# Autodesk Inventor assembly: CNC3
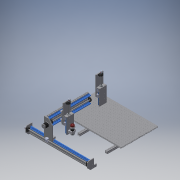
[picture p0: Inventor's stored thumbnail of the model, 180x180]
Saved by Autodesk Inventor 2018 (Build 220112000, 112)
## iProperties
Created: 2018-10-09
Part Number: CNC3
Material: Genérico
Document SubType Name: Assembly
Designer: Georgines
Author: Georgines
## Documents named in this file (29)
- C:\Users\Usuário\Documents\OpenCNC\MONTAGEM\CNC3.iam
- C:\Users\Usuário\Documents\OpenCNC\COMPONENTES_MECANICOS\BLOCOS_GUIAS_LINEARES\SBR16UU.ipt
- C:\Users\Usuário\Documents\OpenCNC\MONTAGEM\CNC1\APOIO_PERFIL_STRUTURAL.ipt
- C:\Users\Usuário\Documents\OpenCNC\MONTAGEM\CNC1\LATERAL_BLOCOS_BASE.ipt
- C:\Users\Usuário\Documents\OpenCNC\MONTAGEM\BLOCO_SUPORTE_EIXO_Z.ipt
- C:\Users\Usuário\Documents\OpenCNC\BAIXADOS\spindle-bldc-500w-1.snapshot.1\SPINDLE_500WSpindle.iam
- C:\Users\Usuário\Documents\OpenCNC\BAIXADOS\spindle-bracket-1.snapshot.2\SUPORTE_SPINDLESpindle Bracket.ipt
- C:\Users\Usuário\Documents\OpenCNC\MONTAGEM\CNC1\BLOCO_SUPORTE_SPINDLE.ipt
- C:\Users\Usuário\Documents\OpenCNC\BAIXADOS\bearing-support-unit-1.snapshot.1\BK12BK12.ipt
- C:\Users\Usuário\Documents\OpenCNC\BAIXADOS\bearing-support-unit-1.snapshot.1\BF12.ipt
- C:\Users\Usuário\Documents\OpenCNC\COMPONENTES_MECANICOS\GUIAS_LINEARES\SBR16_200MM.ipt
- C:\Users\Usuário\Documents\OpenCNC\COMPONENTES_MECANICOS\GUIAS_LINEARES\SBR16_EIXO_X_1.ipt
- C:\Users\Usuário\Documents\OpenCNC\BAIXADOS\stepper motor NEMA 23 57x76.ipt
- C:\Users\Usuário\Documents\OpenCNC\MONTAGEM\CHAPA_APOIO_CASTANHA_EIXO_Z.ipt
- C:\Users\Usuário\Documents\OpenCNC\COMPONENTES_MECANICOS\GUIAS_LINEARES\SBR16_EIXO_Y_1.ipt
- C:\Users\Usuário\Documents\OpenCNC\COMPONENTES_MECANICOS\PERFIL_ESTRUTURAL\PERFIL_ESTRUTURAL_40X80_EIXO_Y.ipt
- C:\Users\Usuário\Documents\OpenCNC\COMPONENTES_MECANICOS\PERFIL_ESTRUTURAL\PERFIL_ESTRUTURAL_40X40_EIXO_Y_PERPENDICULAR.ipt
- C:\Users\Usuário\Documents\OpenCNC\COMPONENTES_MECANICOS\FUSOS\SFU16XX_Y1.ipt
- C:\Users\Usuário\Documents\OpenCNC\COMPONENTES_MECANICOS\FUSOS\SFU16XX_Z.ipt
- C:\Users\Usuário\Documents\OpenCNC\COMPONENTES_MECANICOS\FUSOS\SFU16XX_X.ipt
- C:\Users\Usuário\Documents\OpenCNC\COMPONENTES_MECANICOS\CASTANHAS\CASTANHA_SFU1604SFU1604.ipt
- C:\Users\Usuário\Documents\OpenCNC\COMPONENTES_MECANICOS\ACOPLADORES\ACLOPLADOR_Jaw 6,35x10 d=25 L=30.ipt
- C:\Users\Usuário\Documents\OpenCNC\COMPONENTES_MECANICOS\PERFIL_ESTRUTURAL\PERFIL_ESTRUTURAL_30X60_EIXO_X1.ipt
- C:\Users\Usuário\Documents\OpenCNC\COMPONENTES_MECANICOS\PERFIL_ESTRUTURAL\PERFIL_ESTRUTURAL_30X60_EIXO_X2.ipt
- C:\Users\Usuário\Documents\OpenCNC\COMPONENTES_MECANICOS\SUPORTE_CASTANHAS\SUPORTE_CASTANHAS_DSG16H.ipt
- C:\Users\Usuário\Documents\OpenCNC\MONTAGEM\SUPORTE_MANCAL_FRONTAL.ipt
- C:\Users\Usuário\Documents\OpenCNC\COMPONENTES_MECANICOS\PERFIL_ESTRUTURAL\PERFIL_ESTRUTURAL_20X40_MESA.ipt
- C:\Users\Usuário\Documents\BLOCO_SUPORTE_SPINDLE_E_EIXO_X.ipt
- C:\Users\Usuário\Documents\OpenCNC\MONTAGEM\SUPORTE_MANCAL_TRASEIRO.ipt
## Components (81 placed, 28 different names)
1. SBR16UU:1 — ALINHAMENTO_BOCOS_BASE_4, Alinhamento:32, Coincidência:22, Coincidência:109, Alinhamento:277, Alinhamento:278
2. SBR16UU:2 — ALINHAMENTO_BOCOS_BASE_4, Alinhamento:31, Alinhamento:149, Coincidência:110
3. APOIO_PERFIL_STRUTURAL:1 — Alinhamento:31, Alinhamento:32, Coincidência:22, Alinhamento:85, Alinhamento:149, Alinhamento:177, Coincidência:253, Alinhamento:277, Alinhamento:278
4. LATERAL_BLOCOS_BASE:1 — Alinhamento:85, Alinhamento:177, Coincidência:173, Alinhamento:191, Alinhamento:192, Coincidência:191, Ângulo:3, Alinhamento:200, Ângulo:9, Coincidência:198, Alinhamento:208, Coincidência:253, Alinhamento:275, Alinhamento:276
5. BLOCO_SUPORTE_EIXO_Z:1 — Coincidência:66, Coincidência:77, Alinhamento:118, Alinhamento:122, Alinhamento:124, Coincidência:232, Alinhamento:253, Alinhamento:254
6. SPINDLE_500WSpindle:1 [sub-assembly] — Coincidência:63, Alinhamento:99
7. SUPORTE_SPINDLESpindle Bracket:1 — Coincidência:62, Alinhamento:97, Alinhamento:98, Coincidência:63, Alinhamento:99
8. BLOCO_SUPORTE_SPINDLE:1 — Coincidência:62, Alinhamento:97, Alinhamento:98, Coincidência:79, Coincidência:81, Alinhamento:119, Alinhamento:120, Alinhamento:121, Alinhamento:151, Alinhamento:152, Alinhamento:153
9. BK12BK12:1 — Coincidência:66, Alinhamento:103, Alinhamento:124, Coincidência:181, Coincidência:182, Coincidência:203
10. BF12:1 — Alinhamento:103, Coincidência:180, Coincidência:184, Coincidência:234
11. SBR16UU:9 — Alinhamento:104, Alinhamento:106, Alinhamento:109, Coincidência:75, Coincidência:76, Coincidência:77, Coincidência:78, Alinhamento:122
12. SBR16UU:10 — Alinhamento:104, Alinhamento:107, Alinhamento:108, Alinhamento:109, Coincidência:76, Coincidência:80, Coincidência:234
13. SBR16UU:11 — Alinhamento:105, Alinhamento:106, Alinhamento:110, Coincidência:75
14. SBR16UU:12 — Alinhamento:105, Alinhamento:107, Alinhamento:108, Alinhamento:110, Alinhamento:118
15. SBR16_200MM:1 — Coincidência:78, Coincidência:79, Alinhamento:119, Alinhamento:121
16. SBR16_200MM:2 — Coincidência:80, Coincidência:81, Alinhamento:120
17. SBR16UU:13 — Coincidência:169, Alinhamento:194, Alinhamento:252
18. SBR16UU:14 — Coincidência:168, Alinhamento:190, Alinhamento:195, Alinhamento:249, Alinhamento:250, Alinhamento:251
19. SBR16UU:15 — Alinhamento:173, Coincidência:166, Alinhamento:190, Alinhamento:195
20. stepper motor NEMA 23 57x76:1 — Coincidência:187, Coincidência:188, Coincidência:198, Ângulo:12
21. CHAPA_APOIO_CASTANHA_EIXO_Z:1 — Alinhamento:151, Alinhamento:152, Alinhamento:153, Coincidência:177, Ângulo:1
22. SBR16_EIXO_Y_1:1 — Coincidência:109, Coincidência:110, Coincidência:115, Alinhamento:158, Alinhamento:159, Alinhamento:280
23. PERFIL_ESTRUTURAL_40X80_EIXO_Y:1 — Coincidência:115, Alinhamento:158, Alinhamento:159, Alinhamento:165, Alinhamento:166, Ângulo:9, Alinhamento:203, Alinhamento:205, Alinhamento:279, Coincidência:254, Coincidência:255, Coincidência:256, Alinhamento:283
24. PERFIL_ESTRUTURAL_40X40_EIXO_Y_PERPENDICULAR:1 — Coincidência:210, Alinhamento:247
25. PERFIL_ESTRUTURAL_40X40_EIXO_Y_PERPENDICULAR:2 — Alinhamento:165, Alinhamento:167, Alinhamento:283
26. PERFIL_ESTRUTURAL_40X40_EIXO_Y_PERPENDICULAR:3 — Alinhamento:166, Alinhamento:167
27. stepper motor NEMA 23 57x76:3 — Coincidência:159, Coincidência:160
28. SBR16UU:17 — Alinhamento:173, Coincidência:167, Alinhamento:194, Alinhamento:257
29. SFU16XX_Y1:1 — Coincidência:136, Coincidência:137, Coincidência:138, Coincidência:139, Coincidência:152, Coincidência:155, Coincidência:157
30. SFU16XX_Z:1 — Coincidência:178, Coincidência:179, Coincidência:180, Coincidência:181, Coincidência:182, Coincidência:183, Coincidência:184
31. SFU16XX_X:1 — Coincidência:146, Coincidência:148, Coincidência:149, Coincidência:151, Coincidência:154, Coincidência:175, Coincidência:176
32. BK12BK12:2 — Coincidência:136, Coincidência:137, Alinhamento:178, Ângulo:21
33. BF12:2 — Coincidência:138, Coincidência:139, Alinhamento:178, Alinhamento:203, Coincidência:205, Ângulo:20
34. BK12BK12:4 — Coincidência:146, Alinhamento:180, Coincidência:151, Ângulo:12, Alinhamento:275, Alinhamento:276
35. BF12:4 — Coincidência:148, Coincidência:149, Alinhamento:180, Ângulo:14, Alinhamento:212
36. CASTANHA_SFU1604SFU1604:1 — Coincidência:152, Coincidência:189, Coincidência:190, Ângulo:2
37. CASTANHA_SFU1604SFU1604:3 — Coincidência:154, Coincidência:195, Coincidência:196
38. CASTANHA_SFU1604SFU1604:4 — Coincidência:177, Coincidência:178, Ângulo:1, Coincidência:203
39. ACLOPLADOR_Jaw 6,35x10 d=25 L=30:2 — Coincidência:155, Coincidência:157, Coincidência:159, Coincidência:160
40. ACLOPLADOR_Jaw 6,35x10 d=25 L=30:3 — Coincidência:179, Coincidência:183
41. ACLOPLADOR_Jaw 6,35x10 d=25 L=30:4 — Coincidência:175, Coincidência:176, Coincidência:187, Coincidência:188
42. PERFIL_ESTRUTURAL_30X60_EIXO_X1:1 — Coincidência:163, Alinhamento:183, Alinhamento:184, Alinhamento:187, Alinhamento:188, Coincidência:173, Alinhamento:191, Alinhamento:192, Coincidência:207, Alinhamento:209, Alinhamento:210
43. PERFIL_ESTRUTURAL_30X60_EIXO_X2:1 — Coincidência:164, Alinhamento:185, Alinhamento:186, Alinhamento:187, Alinhamento:188, Coincidência:208, Alinhamento:211
44. SBR16_EIXO_X_1:2 — Coincidência:163, Alinhamento:183, Alinhamento:184, Coincidência:168, Coincidência:169, Ângulo:14
45. SBR16_EIXO_X_1:3 — Coincidência:164, Alinhamento:185, Alinhamento:186, Coincidência:166, Coincidência:167
46. SUPORTE_CASTANHAS_DSG16H:1 — Coincidência:189, Coincidência:190, Ângulo:2, Coincidência:191, Ângulo:3, Alinhamento:200, Coincidência:205, Alinhamento:208
47. SUPORTE_CASTANHAS_DSG16H:3 — Coincidência:195, Coincidência:196, Coincidência:233, Alinhamento:256
48. SUPORTE_MANCAL_FRONTAL:1 — Alinhamento:205, Coincidência:211, Alinhamento:247, Alinhamento:279, Alinhamento:280, Ângulo:20, Alinhamento:281, Alinhamento:282
49. PERFIL_ESTRUTURAL_30X60_EIXO_X1:2 — Coincidência:207, Alinhamento:209, Alinhamento:210, Coincidência:208, Alinhamento:211, Alinhamento:212
50. PERFIL_ESTRUTURAL_20X40_MESA:1 — Coincidência:209, Coincidência:210, Coincidência:211, Alinhamento:213, Alinhamento:214
51. PERFIL_ESTRUTURAL_20X40_MESA:2 — Coincidência:209, Alinhamento:213, Alinhamento:214, Alinhamento:215, Alinhamento:216, Coincidência:213
52. PERFIL_ESTRUTURAL_20X40_MESA:3 — Alinhamento:215, Alinhamento:216, Coincidência:213, Coincidência:214, Alinhamento:217, Alinhamento:218
53. PERFIL_ESTRUTURAL_20X40_MESA:4 — Coincidência:214, Coincidência:215, Alinhamento:217, Alinhamento:218, Coincidência:216, Alinhamento:219, Alinhamento:220
54. PERFIL_ESTRUTURAL_20X40_MESA:5 — Coincidência:215, Coincidência:216, Alinhamento:219, Alinhamento:220, Coincidência:217, Alinhamento:221, Alinhamento:222
55. PERFIL_ESTRUTURAL_20X40_MESA:6 — Coincidência:217, Alinhamento:221, Alinhamento:222, Coincidência:218, Alinhamento:223, Alinhamento:224
56. PERFIL_ESTRUTURAL_20X40_MESA:7 — Coincidência:218, Alinhamento:223, Alinhamento:224, Coincidência:219, Alinhamento:225, Alinhamento:226
57. PERFIL_ESTRUTURAL_20X40_MESA:8 — Coincidência:219, Alinhamento:225, Alinhamento:226, Coincidência:220, Alinhamento:227, Alinhamento:228
58. PERFIL_ESTRUTURAL_20X40_MESA:9 — Coincidência:220, Alinhamento:227, Alinhamento:228, Coincidência:230, Alinhamento:245, Alinhamento:246
59. PERFIL_ESTRUTURAL_20X40_MESA:10 — Coincidência:230, Alinhamento:245, Alinhamento:246
60. PERFIL_ESTRUTURAL_20X40_MESA:11
61. PERFIL_ESTRUTURAL_20X40_MESA:12
62. PERFIL_ESTRUTURAL_20X40_MESA:13
63. PERFIL_ESTRUTURAL_20X40_MESA:14
64. PERFIL_ESTRUTURAL_20X40_MESA:15
65. PERFIL_ESTRUTURAL_20X40_MESA:16
66. BLOCO_SUPORTE_SPINDLE_E_EIXO_X:1 — Alinhamento:249, Alinhamento:250, Alinhamento:251, Alinhamento:252, Coincidência:232, Alinhamento:253, Alinhamento:254, Coincidência:233, Alinhamento:256, Alinhamento:257
67. BLOCO_SUPORTE_EIXO_Z:2
68. BLOCO_SUPORTE_SPINDLE:2
69. BK12BK12:5
70. BF12:5
71. SBR16UU:18
72. SBR16UU:19
73. SBR16UU:20
74. SBR16UU:21
75. SBR16_200MM:3
76. SBR16_200MM:4
77. CHAPA_APOIO_CASTANHA_EIXO_Z:2
78. SFU16XX_Z:2
79. CASTANHA_SFU1604SFU1604:5
80. ACLOPLADOR_Jaw 6,35x10 d=25 L=30:5
81. SUPORTE_MANCAL_TRASEIRO:1 — Coincidência:256, Alinhamento:281, Alinhamento:282, Ângulo:21
## Relationships (228: Flush 118, Mate 101, Angle 9)
- ALINHAMENTO_BOCOS_BASE_4 [Flush]: SBR16UU:1 ↔ SBR16UU:2
- Alinhamento:31 [Flush]: SBR16UU:2 ↔ APOIO_PERFIL_STRUTURAL:1
- Alinhamento:32 [Flush]: SBR16UU:1 ↔ APOIO_PERFIL_STRUTURAL:1
- Coincidência:22 [Mate]: SBR16UU:1 ↔ APOIO_PERFIL_STRUTURAL:1
- Alinhamento:85 [Flush] (-55 mm): APOIO_PERFIL_STRUTURAL:1 ↔ LATERAL_BLOCOS_BASE:1
- Coincidência:62 [Mate]: SUPORTE_SPINDLESpindle Bracket:1 ↔ BLOCO_SUPORTE_SPINDLE:1
- Alinhamento:97 [Flush] (25 mm): SUPORTE_SPINDLESpindle Bracket:1 ↔ BLOCO_SUPORTE_SPINDLE:1
- Alinhamento:98 [Flush] (18 mm): SUPORTE_SPINDLESpindle Bracket:1 ↔ BLOCO_SUPORTE_SPINDLE:1
- Coincidência:63 [Mate]: SPINDLE_500WSpindle:1 ↔ SUPORTE_SPINDLESpindle Bracket:1
- Alinhamento:99 [Flush] (-25 mm): SPINDLE_500WSpindle:1 ↔ SUPORTE_SPINDLESpindle Bracket:1
- Coincidência:66 [Mate]: BLOCO_SUPORTE_EIXO_Z:1 ↔ BK12BK12:1
- Alinhamento:103 [Flush]: BK12BK12:1 ↔ BF12:1
- Alinhamento:104 [Flush]: SBR16UU:9 ↔ SBR16UU:10
- Alinhamento:105 [Flush]: SBR16UU:11 ↔ SBR16UU:12
- Alinhamento:106 [Flush]: SBR16UU:9 ↔ SBR16UU:11
- Alinhamento:107 [Flush]: SBR16UU:10 ↔ SBR16UU:12
- Alinhamento:108 [Flush]: SBR16UU:10 ↔ SBR16UU:12
- Alinhamento:109 [Flush]: SBR16UU:9 ↔ SBR16UU:10
- Alinhamento:110 [Flush]: SBR16UU:11 ↔ SBR16UU:12
- Coincidência:75 [Mate] (43 mm): SBR16UU:9 ↔ SBR16UU:11
- Coincidência:76 [Mate] (35 mm): SBR16UU:9 ↔ SBR16UU:10
- Coincidência:77 [Mate]: BLOCO_SUPORTE_EIXO_Z:1 ↔ SBR16UU:9
- Alinhamento:118 [Flush]: BLOCO_SUPORTE_EIXO_Z:1 ↔ SBR16UU:12
- Coincidência:78 [Mate]: SBR16UU:9 ↔ SBR16_200MM:1
- Coincidência:79 [Mate]: BLOCO_SUPORTE_SPINDLE:1 ↔ SBR16_200MM:1
- Coincidência:80 [Mate]: SBR16UU:10 ↔ SBR16_200MM:2
- Coincidência:81 [Mate]: BLOCO_SUPORTE_SPINDLE:1 ↔ SBR16_200MM:2
- Alinhamento:119 [Flush]: BLOCO_SUPORTE_SPINDLE:1 ↔ SBR16_200MM:1
- Alinhamento:120 [Flush]: BLOCO_SUPORTE_SPINDLE:1 ↔ SBR16_200MM:2
- Alinhamento:121 [Flush] (-2.5 mm): BLOCO_SUPORTE_SPINDLE:1 ↔ SBR16_200MM:1
- Alinhamento:122 [Flush]: BLOCO_SUPORTE_EIXO_Z:1 ↔ SBR16UU:9
- Alinhamento:124 [Flush] (32.5 mm): BLOCO_SUPORTE_EIXO_Z:1 ↔ BK12BK12:1
- Alinhamento:149 [Flush]: SBR16UU:2 ↔ APOIO_PERFIL_STRUTURAL:1
- Alinhamento:151 [Flush]: BLOCO_SUPORTE_SPINDLE:1 ↔ CHAPA_APOIO_CASTANHA_EIXO_Z:1
- Alinhamento:152 [Flush]: BLOCO_SUPORTE_SPINDLE:1 ↔ CHAPA_APOIO_CASTANHA_EIXO_Z:1
- Alinhamento:153 [Flush]: BLOCO_SUPORTE_SPINDLE:1 ↔ CHAPA_APOIO_CASTANHA_EIXO_Z:1
- Coincidência:109 [Mate]: SBR16UU:1 ↔ SBR16_EIXO_Y_1:1
- Coincidência:110 [Mate]: SBR16UU:2 ↔ SBR16_EIXO_Y_1:1
- Coincidência:115 [Mate]: SBR16_EIXO_Y_1:1 ↔ PERFIL_ESTRUTURAL_40X80_EIXO_Y:1
- Alinhamento:158 [Flush]: SBR16_EIXO_Y_1:1 ↔ PERFIL_ESTRUTURAL_40X80_EIXO_Y:1
- Alinhamento:159 [Flush]: SBR16_EIXO_Y_1:1 ↔ PERFIL_ESTRUTURAL_40X80_EIXO_Y:1
- Alinhamento:165 [Flush]: PERFIL_ESTRUTURAL_40X80_EIXO_Y:1 ↔ PERFIL_ESTRUTURAL_40X40_EIXO_Y_PERPENDICULAR:2
- Alinhamento:166 [Flush]: PERFIL_ESTRUTURAL_40X80_EIXO_Y:1 ↔ PERFIL_ESTRUTURAL_40X40_EIXO_Y_PERPENDICULAR:3
- Alinhamento:167 [Flush] (-433.419 mm): PERFIL_ESTRUTURAL_40X40_EIXO_Y_PERPENDICULAR:2 ↔ PERFIL_ESTRUTURAL_40X40_EIXO_Y_PERPENDICULAR:3
- Alinhamento:173 [Flush]: SBR16UU:15 ↔ SBR16UU:17
- Alinhamento:177 [Flush]: APOIO_PERFIL_STRUTURAL:1 ↔ LATERAL_BLOCOS_BASE:1
- Coincidência:136 [Mate]: SFU16XX_Y1:1 ↔ BK12BK12:2
- Coincidência:137 [Mate]: SFU16XX_Y1:1 ↔ BK12BK12:2
- Coincidência:138 [Mate]: SFU16XX_Y1:1 ↔ BF12:2
- Coincidência:139 [Mate]: SFU16XX_Y1:1 ↔ BF12:2
- Alinhamento:178 [Flush]: BK12BK12:2 ↔ BF12:2
- Coincidência:146 [Mate]: SFU16XX_X:1 ↔ BK12BK12:4
- Coincidência:148 [Mate]: SFU16XX_X:1 ↔ BF12:4
- Coincidência:149 [Mate]: SFU16XX_X:1 ↔ BF12:4
- Alinhamento:180 [Flush]: BK12BK12:4 ↔ BF12:4
- Coincidência:151 [Mate]: SFU16XX_X:1 ↔ BK12BK12:4
- Coincidência:152 [Mate]: SFU16XX_Y1:1 ↔ CASTANHA_SFU1604SFU1604:1
- Coincidência:154 [Mate]: SFU16XX_X:1 ↔ CASTANHA_SFU1604SFU1604:3
- Coincidência:155 [Mate]: SFU16XX_Y1:1 ↔ ACLOPLADOR_Jaw 6,35x10 d=25 L=30:2
- Coincidência:157 [Mate]: SFU16XX_Y1:1 ↔ ACLOPLADOR_Jaw 6,35x10 d=25 L=30:2
- Coincidência:159 [Mate]: stepper motor NEMA 23 57x76:3 ↔ ACLOPLADOR_Jaw 6,35x10 d=25 L=30:2
- Coincidência:160 [Mate] (-15 mm): stepper motor NEMA 23 57x76:3 ↔ ACLOPLADOR_Jaw 6,35x10 d=25 L=30:2
- Coincidência:163 [Mate]: PERFIL_ESTRUTURAL_30X60_EIXO_X1:1 ↔ SBR16_EIXO_X_1:2
- Alinhamento:183 [Flush]: PERFIL_ESTRUTURAL_30X60_EIXO_X1:1 ↔ SBR16_EIXO_X_1:2
- Alinhamento:184 [Flush] (-10 mm): PERFIL_ESTRUTURAL_30X60_EIXO_X1:1 ↔ SBR16_EIXO_X_1:2
- Coincidência:164 [Mate]: PERFIL_ESTRUTURAL_30X60_EIXO_X2:1 ↔ SBR16_EIXO_X_1:3
- Alinhamento:185 [Flush]: PERFIL_ESTRUTURAL_30X60_EIXO_X2:1 ↔ SBR16_EIXO_X_1:3
- Alinhamento:186 [Flush] (10 mm): PERFIL_ESTRUTURAL_30X60_EIXO_X2:1 ↔ SBR16_EIXO_X_1:3
- Alinhamento:187 [Flush]: PERFIL_ESTRUTURAL_30X60_EIXO_X1:1 ↔ PERFIL_ESTRUTURAL_30X60_EIXO_X2:1
- Alinhamento:188 [Flush]: PERFIL_ESTRUTURAL_30X60_EIXO_X1:1 ↔ PERFIL_ESTRUTURAL_30X60_EIXO_X2:1
- Coincidência:166 [Mate]: SBR16UU:15 ↔ SBR16_EIXO_X_1:3
- Coincidência:167 [Mate]: SBR16UU:17 ↔ SBR16_EIXO_X_1:3
- Coincidência:168 [Mate]: SBR16UU:14 ↔ SBR16_EIXO_X_1:2
- Coincidência:169 [Mate]: SBR16UU:13 ↔ SBR16_EIXO_X_1:2
- Alinhamento:190 [Flush]: SBR16UU:14 ↔ SBR16UU:15
- Coincidência:173 [Mate]: LATERAL_BLOCOS_BASE:1 ↔ PERFIL_ESTRUTURAL_30X60_EIXO_X1:1
- Alinhamento:191 [Flush] (10 mm): LATERAL_BLOCOS_BASE:1 ↔ PERFIL_ESTRUTURAL_30X60_EIXO_X1:1
- Alinhamento:192 [Flush]: LATERAL_BLOCOS_BASE:1 ↔ PERFIL_ESTRUTURAL_30X60_EIXO_X1:1
- Coincidência:175 [Mate]: SFU16XX_X:1 ↔ ACLOPLADOR_Jaw 6,35x10 d=25 L=30:4
- Coincidência:176 [Mate] (-15 mm): SFU16XX_X:1 ↔ ACLOPLADOR_Jaw 6,35x10 d=25 L=30:4
- Coincidência:177 [Mate]: CHAPA_APOIO_CASTANHA_EIXO_Z:1 ↔ CASTANHA_SFU1604SFU1604:4
- Coincidência:178 [Mate]: SFU16XX_Z:1 ↔ CASTANHA_SFU1604SFU1604:4
- Coincidência:179 [Mate]: SFU16XX_Z:1 ↔ ACLOPLADOR_Jaw 6,35x10 d=25 L=30:3
- Coincidência:180 [Mate]: BF12:1 ↔ SFU16XX_Z:1
- Coincidência:181 [Mate]: BK12BK12:1 ↔ SFU16XX_Z:1
- Coincidência:182 [Mate]: BK12BK12:1 ↔ SFU16XX_Z:1
- Ângulo:1 [Angle] (0 deg): CHAPA_APOIO_CASTANHA_EIXO_Z:1 ↔ CASTANHA_SFU1604SFU1604:4
- Coincidência:183 [Mate] (-15 mm): SFU16XX_Z:1 ↔ ACLOPLADOR_Jaw 6,35x10 d=25 L=30:3
- Coincidência:184 [Mate]: BF12:1 ↔ SFU16XX_Z:1
- Alinhamento:194 [Flush]: SBR16UU:13 ↔ SBR16UU:17
- Alinhamento:195 [Flush]: SBR16UU:14 ↔ SBR16UU:15
- Coincidência:187 [Mate]: stepper motor NEMA 23 57x76:1 ↔ ACLOPLADOR_Jaw 6,35x10 d=25 L=30:4
- Coincidência:188 [Mate] (-15 mm): stepper motor NEMA 23 57x76:1 ↔ ACLOPLADOR_Jaw 6,35x10 d=25 L=30:4
- Coincidência:189 [Mate]: CASTANHA_SFU1604SFU1604:1 ↔ SUPORTE_CASTANHAS_DSG16H:1
- Coincidência:190 [Mate]: CASTANHA_SFU1604SFU1604:1 ↔ SUPORTE_CASTANHAS_DSG16H:1
- Ângulo:2 [Angle] (0 deg): CASTANHA_SFU1604SFU1604:1 ↔ SUPORTE_CASTANHAS_DSG16H:1
- Coincidência:191 [Mate]: LATERAL_BLOCOS_BASE:1 ↔ SUPORTE_CASTANHAS_DSG16H:1
- Ângulo:3 [Angle] (0 deg): LATERAL_BLOCOS_BASE:1 ↔ SUPORTE_CASTANHAS_DSG16H:1
- Alinhamento:200 [Flush] (-50 mm): LATERAL_BLOCOS_BASE:1 ↔ SUPORTE_CASTANHAS_DSG16H:1
- Ângulo:9 [Angle] (0 deg): LATERAL_BLOCOS_BASE:1 ↔ PERFIL_ESTRUTURAL_40X80_EIXO_Y:1
- Coincidência:195 [Mate]: CASTANHA_SFU1604SFU1604:3 ↔ SUPORTE_CASTANHAS_DSG16H:3
- Coincidência:196 [Mate]: CASTANHA_SFU1604SFU1604:3 ↔ SUPORTE_CASTANHAS_DSG16H:3
- Coincidência:198 [Mate]: LATERAL_BLOCOS_BASE:1 ↔ stepper motor NEMA 23 57x76:1
- Ângulo:12 [Angle] (0 deg): stepper motor NEMA 23 57x76:1 ↔ BK12BK12:4
- Ângulo:14 [Angle] (0 deg): BF12:4 ↔ SBR16_EIXO_X_1:2
- Coincidência:203 [Mate] (155 mm): BK12BK12:1 ↔ CASTANHA_SFU1604SFU1604:4
- Alinhamento:203 [Flush]: PERFIL_ESTRUTURAL_40X80_EIXO_Y:1 ↔ BF12:2
- Coincidência:205 [Mate]: BF12:2 ↔ SUPORTE_CASTANHAS_DSG16H:1
- Alinhamento:205 [Flush]: PERFIL_ESTRUTURAL_40X80_EIXO_Y:1 ↔ SUPORTE_MANCAL_FRONTAL:1
- Alinhamento:208 [Flush]: LATERAL_BLOCOS_BASE:1 ↔ SUPORTE_CASTANHAS_DSG16H:1
- Coincidência:207 [Mate]: PERFIL_ESTRUTURAL_30X60_EIXO_X1:1 ↔ PERFIL_ESTRUTURAL_30X60_EIXO_X1:2
- Alinhamento:209 [Flush]: PERFIL_ESTRUTURAL_30X60_EIXO_X1:1 ↔ PERFIL_ESTRUTURAL_30X60_EIXO_X1:2
- Alinhamento:210 [Flush]: PERFIL_ESTRUTURAL_30X60_EIXO_X1:1 ↔ PERFIL_ESTRUTURAL_30X60_EIXO_X1:2
- Coincidência:208 [Mate]: PERFIL_ESTRUTURAL_30X60_EIXO_X2:1 ↔ PERFIL_ESTRUTURAL_30X60_EIXO_X1:2
- Alinhamento:211 [Flush]: PERFIL_ESTRUTURAL_30X60_EIXO_X2:1 ↔ PERFIL_ESTRUTURAL_30X60_EIXO_X1:2
- Alinhamento:212 [Flush]: BF12:4 ↔ PERFIL_ESTRUTURAL_30X60_EIXO_X1:2
- Coincidência:209 [Mate]: PERFIL_ESTRUTURAL_20X40_MESA:1 ↔ PERFIL_ESTRUTURAL_20X40_MESA:2
- Coincidência:210 [Mate]: PERFIL_ESTRUTURAL_40X40_EIXO_Y_PERPENDICULAR:1 ↔ PERFIL_ESTRUTURAL_20X40_MESA:1
- Coincidência:211 [Mate]: SUPORTE_MANCAL_FRONTAL:1 ↔ PERFIL_ESTRUTURAL_20X40_MESA:1
- Alinhamento:213 [Flush]: PERFIL_ESTRUTURAL_20X40_MESA:1 ↔ PERFIL_ESTRUTURAL_20X40_MESA:2
- Alinhamento:214 [Flush]: PERFIL_ESTRUTURAL_20X40_MESA:1 ↔ PERFIL_ESTRUTURAL_20X40_MESA:2
- Alinhamento:215 [Flush]: PERFIL_ESTRUTURAL_20X40_MESA:2 ↔ PERFIL_ESTRUTURAL_20X40_MESA:3
- Alinhamento:216 [Flush]: PERFIL_ESTRUTURAL_20X40_MESA:2 ↔ PERFIL_ESTRUTURAL_20X40_MESA:3
- Coincidência:213 [Mate]: PERFIL_ESTRUTURAL_20X40_MESA:2 ↔ PERFIL_ESTRUTURAL_20X40_MESA:3
- Coincidência:214 [Mate]: PERFIL_ESTRUTURAL_20X40_MESA:3 ↔ PERFIL_ESTRUTURAL_20X40_MESA:4
- Coincidência:215 [Mate]: PERFIL_ESTRUTURAL_20X40_MESA:4 ↔ PERFIL_ESTRUTURAL_20X40_MESA:5
- Alinhamento:217 [Flush]: PERFIL_ESTRUTURAL_20X40_MESA:3 ↔ PERFIL_ESTRUTURAL_20X40_MESA:4
- Alinhamento:218 [Flush]: PERFIL_ESTRUTURAL_20X40_MESA:3 ↔ PERFIL_ESTRUTURAL_20X40_MESA:4
- Coincidência:216 [Mate]: PERFIL_ESTRUTURAL_20X40_MESA:4 ↔ PERFIL_ESTRUTURAL_20X40_MESA:5
- Alinhamento:219 [Flush]: PERFIL_ESTRUTURAL_20X40_MESA:4 ↔ PERFIL_ESTRUTURAL_20X40_MESA:5
- Alinhamento:220 [Flush]: PERFIL_ESTRUTURAL_20X40_MESA:4 ↔ PERFIL_ESTRUTURAL_20X40_MESA:5
- Coincidência:217 [Mate]: PERFIL_ESTRUTURAL_20X40_MESA:5 ↔ PERFIL_ESTRUTURAL_20X40_MESA:6
- Alinhamento:221 [Flush]: PERFIL_ESTRUTURAL_20X40_MESA:5 ↔ PERFIL_ESTRUTURAL_20X40_MESA:6
- Alinhamento:222 [Flush]: PERFIL_ESTRUTURAL_20X40_MESA:5 ↔ PERFIL_ESTRUTURAL_20X40_MESA:6
- Coincidência:218 [Mate]: PERFIL_ESTRUTURAL_20X40_MESA:6 ↔ PERFIL_ESTRUTURAL_20X40_MESA:7
- Alinhamento:223 [Flush]: PERFIL_ESTRUTURAL_20X40_MESA:6 ↔ PERFIL_ESTRUTURAL_20X40_MESA:7
- Alinhamento:224 [Flush]: PERFIL_ESTRUTURAL_20X40_MESA:6 ↔ PERFIL_ESTRUTURAL_20X40_MESA:7
- Coincidência:219 [Mate]: PERFIL_ESTRUTURAL_20X40_MESA:7 ↔ PERFIL_ESTRUTURAL_20X40_MESA:8
- Alinhamento:225 [Flush]: PERFIL_ESTRUTURAL_20X40_MESA:7 ↔ PERFIL_ESTRUTURAL_20X40_MESA:8
- Alinhamento:226 [Flush]: PERFIL_ESTRUTURAL_20X40_MESA:7 ↔ PERFIL_ESTRUTURAL_20X40_MESA:8
- Coincidência:220 [Mate]: PERFIL_ESTRUTURAL_20X40_MESA:8 ↔ PERFIL_ESTRUTURAL_20X40_MESA:9
- Alinhamento:227 [Flush]: PERFIL_ESTRUTURAL_20X40_MESA:8 ↔ PERFIL_ESTRUTURAL_20X40_MESA:9
- Alinhamento:228 [Flush]: PERFIL_ESTRUTURAL_20X40_MESA:8 ↔ PERFIL_ESTRUTURAL_20X40_MESA:9
- [Mate]: PERFIL_ESTRUTURAL_20X40_MESA:10 ↔ PERFIL_ESTRUTURAL_20X40_MESA:11
- [Flush]: PERFIL_ESTRUTURAL_20X40_MESA:10 ↔ PERFIL_ESTRUTURAL_20X40_MESA:11
- [Flush]: PERFIL_ESTRUTURAL_20X40_MESA:10 ↔ PERFIL_ESTRUTURAL_20X40_MESA:11
- [Flush]: PERFIL_ESTRUTURAL_20X40_MESA:11 ↔ PERFIL_ESTRUTURAL_20X40_MESA:12
- [Flush]: PERFIL_ESTRUTURAL_20X40_MESA:11 ↔ PERFIL_ESTRUTURAL_20X40_MESA:12
- [Mate]: PERFIL_ESTRUTURAL_20X40_MESA:11 ↔ PERFIL_ESTRUTURAL_20X40_MESA:12
- [Mate]: PERFIL_ESTRUTURAL_20X40_MESA:12 ↔ PERFIL_ESTRUTURAL_20X40_MESA:13
- [Mate]: PERFIL_ESTRUTURAL_20X40_MESA:13 ↔ PERFIL_ESTRUTURAL_20X40_MESA:14
- [Flush]: PERFIL_ESTRUTURAL_20X40_MESA:12 ↔ PERFIL_ESTRUTURAL_20X40_MESA:13
- [Flush]: PERFIL_ESTRUTURAL_20X40_MESA:12 ↔ PERFIL_ESTRUTURAL_20X40_MESA:13
- [Mate]: PERFIL_ESTRUTURAL_20X40_MESA:13 ↔ PERFIL_ESTRUTURAL_20X40_MESA:14
- [Flush]: PERFIL_ESTRUTURAL_20X40_MESA:13 ↔ PERFIL_ESTRUTURAL_20X40_MESA:14
- [Flush]: PERFIL_ESTRUTURAL_20X40_MESA:13 ↔ PERFIL_ESTRUTURAL_20X40_MESA:14
- [Mate]: PERFIL_ESTRUTURAL_20X40_MESA:14 ↔ PERFIL_ESTRUTURAL_20X40_MESA:15
- [Flush]: PERFIL_ESTRUTURAL_20X40_MESA:14 ↔ PERFIL_ESTRUTURAL_20X40_MESA:15
- [Flush]: PERFIL_ESTRUTURAL_20X40_MESA:14 ↔ PERFIL_ESTRUTURAL_20X40_MESA:15
- [Mate]: PERFIL_ESTRUTURAL_20X40_MESA:15 ↔ PERFIL_ESTRUTURAL_20X40_MESA:16
- [Flush]: PERFIL_ESTRUTURAL_20X40_MESA:15 ↔ PERFIL_ESTRUTURAL_20X40_MESA:16
- [Flush]: PERFIL_ESTRUTURAL_20X40_MESA:15 ↔ PERFIL_ESTRUTURAL_20X40_MESA:16
- Coincidência:230 [Mate]: PERFIL_ESTRUTURAL_20X40_MESA:9 ↔ PERFIL_ESTRUTURAL_20X40_MESA:10
- Alinhamento:245 [Flush]: PERFIL_ESTRUTURAL_20X40_MESA:9 ↔ PERFIL_ESTRUTURAL_20X40_MESA:10
- Alinhamento:246 [Flush]: PERFIL_ESTRUTURAL_20X40_MESA:9 ↔ PERFIL_ESTRUTURAL_20X40_MESA:10
- Alinhamento:247 [Flush]: PERFIL_ESTRUTURAL_40X40_EIXO_Y_PERPENDICULAR:1 ↔ SUPORTE_MANCAL_FRONTAL:1
- Alinhamento:249 [Flush]: SBR16UU:14 ↔ BLOCO_SUPORTE_SPINDLE_E_EIXO_X:1
- Alinhamento:250 [Flush]: SBR16UU:14 ↔ BLOCO_SUPORTE_SPINDLE_E_EIXO_X:1
- Alinhamento:251 [Flush] (20 mm): SBR16UU:14 ↔ BLOCO_SUPORTE_SPINDLE_E_EIXO_X:1
- Alinhamento:252 [Flush]: SBR16UU:13 ↔ BLOCO_SUPORTE_SPINDLE_E_EIXO_X:1
- Coincidência:232 [Mate]: BLOCO_SUPORTE_EIXO_Z:1 ↔ BLOCO_SUPORTE_SPINDLE_E_EIXO_X:1
- Alinhamento:253 [Flush]: BLOCO_SUPORTE_EIXO_Z:1 ↔ BLOCO_SUPORTE_SPINDLE_E_EIXO_X:1
- Alinhamento:254 [Flush]: BLOCO_SUPORTE_EIXO_Z:1 ↔ BLOCO_SUPORTE_SPINDLE_E_EIXO_X:1
- Coincidência:233 [Mate]: SUPORTE_CASTANHAS_DSG16H:3 ↔ BLOCO_SUPORTE_SPINDLE_E_EIXO_X:1
- Alinhamento:256 [Flush] (42.5 mm): SUPORTE_CASTANHAS_DSG16H:3 ↔ BLOCO_SUPORTE_SPINDLE_E_EIXO_X:1
- Alinhamento:257 [Flush]: SBR16UU:17 ↔ BLOCO_SUPORTE_SPINDLE_E_EIXO_X:1
- Coincidência:234 [Mate] (14.03 mm): BF12:1 ↔ SBR16UU:10
- [Mate]: BLOCO_SUPORTE_EIXO_Z:2 ↔ BK12BK12:5
- [Flush]: BK12BK12:5 ↔ BF12:5
- [Flush]: SBR16UU:18 ↔ SBR16UU:19
- [Flush]: SBR16UU:20 ↔ SBR16UU:21
- [Flush]: SBR16UU:18 ↔ SBR16UU:20
- [Flush]: SBR16UU:19 ↔ SBR16UU:21
- [Flush]: SBR16UU:19 ↔ SBR16UU:21
- [Flush]: SBR16UU:18 ↔ SBR16UU:19
- [Flush]: SBR16UU:20 ↔ SBR16UU:21
- [Mate] (43 mm): SBR16UU:18 ↔ SBR16UU:20
- [Mate] (35 mm): SBR16UU:18 ↔ SBR16UU:19
- [Mate]: BLOCO_SUPORTE_EIXO_Z:2 ↔ SBR16UU:18
- [Flush]: BLOCO_SUPORTE_EIXO_Z:2 ↔ SBR16UU:21
- [Mate]: SBR16UU:18 ↔ SBR16_200MM:3
- [Mate]: BLOCO_SUPORTE_SPINDLE:2 ↔ SBR16_200MM:3
- [Mate]: SBR16UU:19 ↔ SBR16_200MM:4
- [Mate]: BLOCO_SUPORTE_SPINDLE:2 ↔ SBR16_200MM:4
- [Flush]: BLOCO_SUPORTE_SPINDLE:2 ↔ SBR16_200MM:3
- [Flush]: BLOCO_SUPORTE_SPINDLE:2 ↔ SBR16_200MM:4
- [Flush] (-2.5 mm): BLOCO_SUPORTE_SPINDLE:2 ↔ SBR16_200MM:3
- [Flush]: BLOCO_SUPORTE_EIXO_Z:2 ↔ SBR16UU:18
- [Flush] (32.5 mm): BLOCO_SUPORTE_EIXO_Z:2 ↔ BK12BK12:5
- [Flush]: BLOCO_SUPORTE_SPINDLE:2 ↔ CHAPA_APOIO_CASTANHA_EIXO_Z:2
- [Flush]: BLOCO_SUPORTE_SPINDLE:2 ↔ CHAPA_APOIO_CASTANHA_EIXO_Z:2
- [Flush]: BLOCO_SUPORTE_SPINDLE:2 ↔ CHAPA_APOIO_CASTANHA_EIXO_Z:2
- [Mate]: CHAPA_APOIO_CASTANHA_EIXO_Z:2 ↔ CASTANHA_SFU1604SFU1604:5
- [Mate]: SFU16XX_Z:2 ↔ CASTANHA_SFU1604SFU1604:5
- [Mate]: SFU16XX_Z:2 ↔ ACLOPLADOR_Jaw 6,35x10 d=25 L=30:5
- [Mate]: BF12:5 ↔ SFU16XX_Z:2
- [Mate]: BK12BK12:5 ↔ SFU16XX_Z:2
- [Mate]: BK12BK12:5 ↔ SFU16XX_Z:2
- [Angle] (0 deg): CHAPA_APOIO_CASTANHA_EIXO_Z:2 ↔ CASTANHA_SFU1604SFU1604:5
- [Mate] (-15 mm): SFU16XX_Z:2 ↔ ACLOPLADOR_Jaw 6,35x10 d=25 L=30:5
- [Mate]: BF12:5 ↔ SFU16XX_Z:2
- [Mate] (155 mm): BK12BK12:5 ↔ CASTANHA_SFU1604SFU1604:5
- [Mate] (14.03 mm): BF12:5 ↔ SBR16UU:19
- Coincidência:253 [Mate]: APOIO_PERFIL_STRUTURAL:1 ↔ LATERAL_BLOCOS_BASE:1
- Alinhamento:275 [Flush] (60 mm): LATERAL_BLOCOS_BASE:1 ↔ BK12BK12:4
- Alinhamento:276 [Flush] (57 mm): LATERAL_BLOCOS_BASE:1 ↔ BK12BK12:4
- Alinhamento:277 [Flush]: SBR16UU:1 ↔ APOIO_PERFIL_STRUTURAL:1
- Alinhamento:278 [Flush]: SBR16UU:1 ↔ APOIO_PERFIL_STRUTURAL:1
- Alinhamento:279 [Flush] (-63.5 mm): PERFIL_ESTRUTURAL_40X80_EIXO_Y:1 ↔ SUPORTE_MANCAL_FRONTAL:1
- Alinhamento:280 [Flush] (-60 mm): SBR16_EIXO_Y_1:1 ↔ SUPORTE_MANCAL_FRONTAL:1
- Coincidência:254 [Mate] (28.28 mm): PERFIL_ESTRUTURAL_40X80_EIXO_Y:1
- Coincidência:255 [Mate]: PERFIL_ESTRUTURAL_40X80_EIXO_Y:1
- Ângulo:20 [Angle] (0 deg): BF12:2 ↔ SUPORTE_MANCAL_FRONTAL:1
- Coincidência:256 [Mate]: PERFIL_ESTRUTURAL_40X80_EIXO_Y:1 ↔ SUPORTE_MANCAL_TRASEIRO:1
- Alinhamento:281 [Flush]: SUPORTE_MANCAL_FRONTAL:1 ↔ SUPORTE_MANCAL_TRASEIRO:1
- Alinhamento:282 [Flush]: SUPORTE_MANCAL_FRONTAL:1 ↔ SUPORTE_MANCAL_TRASEIRO:1
- Ângulo:21 [Angle] (0 deg): BK12BK12:2 ↔ SUPORTE_MANCAL_TRASEIRO:1
- Alinhamento:283 [Flush]: PERFIL_ESTRUTURAL_40X80_EIXO_Y:1 ↔ PERFIL_ESTRUTURAL_40X40_EIXO_Y_PERPENDICULAR:2
## Named parameters: d552_d524 = 0 mm, d553_d528 = 0 mm, d554_d543 = 0 mm, d555_d544 = 0 mm, d556_d545 = 0 mm, d563_d529 = 0 mm, d564_d530 = 0 mm, d565_d531 = 0 mm, d566_d532 = 0 mm, d567_d533 = 0 mm, d568_d534 = 0 mm, d569_d535 = 0 mm, d570_d536 = 0 mm, d571_d537 = 0 mm, d572_d538 = 0 mm, d573_d539 = 0 mm, d574_d540 = 0 mm, d575_d541 = 0 mm, d576_d542 = 0 mm, d626_d594 = 14.03 mm, d627_d496 = 155 mm, d628_d497 = 149 mm, d629_d498 = 5 mm, d630_d440 = 0 mm, d631_d441 = 0 mm, d632_d442 = 0 mm, d633_d443 = 0 mm, d634_d445 = 0 mm, d635_d446 = 0 mm, d636_d447 = 0 deg, d637_d448 = -15 mm, d638_d449 = 0 mm, d639_d220 = 32.5 mm, d640_d295 = 0 mm, d641_d296 = 0 mm, d642_d297 = 0 mm, d643_d172 = 0 mm, d644_d184 = 0 mm, d645_d186 = 0 mm, d646_d187 = 0 mm, d647_d188 = 0 mm, d648_d189 = 0 mm, d649_d190 = 0 mm, d650_d191 = 0 mm, d651_d192 = 0 mm, d652_d193 = 43 mm, d653_d194 = 35 mm, d654_d195 = 0 mm, d655_d209 = 0 mm, d656_d210 = 0 mm, d657_d211 = 0 mm, d658_d212 = 0 mm, d659_d213 = 0 mm, d660_d214 = 0 mm, d661_d215 = 0 mm, d662_d216 = -2.5 mm, d663_d217 = 0 mm
